# Autodesk Inventor assembly: 1段目
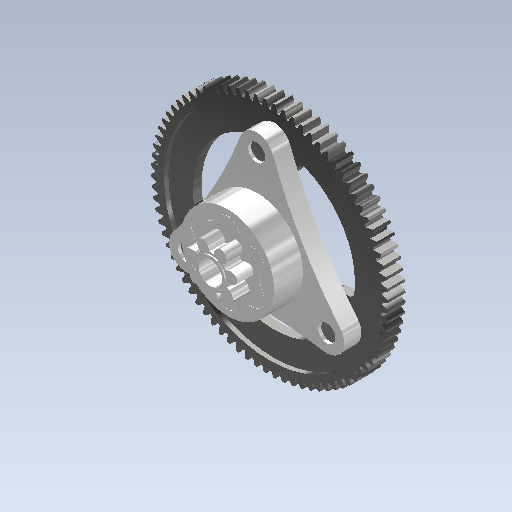
[picture p0: Inventor's stored thumbnail of the model, 512x512]
Saved by Autodesk Inventor 2020.4 (Build 244396000, 396)
## iProperties
Created: 2021-04-23
Part Number: 1段目
Document SubType Name: Assembly
Designer: happy
Mass: 18.9935 g
Surface Area: 61.5012 cm^2
Volume: 4.00861 cm^3
Density: 4.73818 g/cm^3
Author: happy
## Documents named in this file (6)
- C:\Users\happy\OneDrive\ドキュメント\賢一ファイル\SRDC\試作10-2\アームギア\1段目.iam
- C:\Users\happy\OneDrive\ドキュメント\賢一ファイル\SRDC\試作10-2\アームギア\1ギア接続部.ipt
- C:\Users\happy\OneDrive\ドキュメント\賢一ファイル\SRDC\試作10-2\アームギア\1ギア接続部外.ipt
- C:\Users\happy\OneDrive\ドキュメント\賢一ファイル\SRDC\試作10-2\アームギア\m0.5z80.iam
- C:\Users\happy\OneDrive\ドキュメント\賢一ファイル\SRDC\試作10-2\アームギア\m1z7.ipt
- C:\Users\happy\OneDrive\ドキュメント\賢一ファイル\SRDC\試作10-2\アームギア\1ギア補強材.ipt
## Components (5 placed, 5 different names)
1. 1ギア接続部:1 — 挿入:1, 挿入:2, 挿入:6, メイト:2
2. 1ギア接続部外:1 — メイト:1, メイト:3, フラッシュ:1
3. m0.5z80:1 [sub-assembly] — 挿入:1, 挿入:5, メイト:2
4. m1z7:1 — 挿入:2, メイト:1, 挿入:6, メイト:3, フラッシュ:1
5. 1ギア補強材:1 — 挿入:5
## Relationships (8: Insert 4, Mate 3, Flush 1)
- 挿入:1 [Insert]: 1ギア接続部:1 ↔ m0.5z80:1
- 挿入:2 [Insert]: 1ギア接続部:1 ↔ m1z7:1
- メイト:1 [Mate]: 1ギア接続部外:1 ↔ m1z7:1
- 挿入:5 [Insert]: m0.5z80:1 ↔ 1ギア補強材:1
- 挿入:6 [Insert]: 1ギア接続部:1 ↔ m1z7:1
- メイト:2 [Mate]: 1ギア接続部:1 ↔ m0.5z80:1
- メイト:3 [Mate]: 1ギア接続部外:1 ↔ m1z7:1
- フラッシュ:1 [Flush]: 1ギア接続部外:1 ↔ m1z7:1
